# Autodesk Inventor assembly: functioning swerve drive
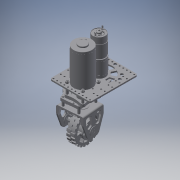
[picture p0: Inventor's stored thumbnail of the model, 180x180]
Saved by Autodesk Inventor 2019 (Build 230136000, 136)
## iProperties
Created: 2019-01-14
Part Number: functioning swerve drive
Document SubType Name: Assembly
Designer: josh
Author: josh
## Documents named in this file (35)
- D:\Synthesis Robots\Epsilon\Functioning swerve drive sub-assemblies\functioning swerve drive.iam
- D:\Synthesis Robots\Epsilon\Swerve drive parts\FR6ZZ-L Hex Bearing.ipt
- D:\Synthesis Robots\Epsilon\Swerve drive parts\375 Hex Output Shaft Rev 2.ipt
- D:\Synthesis Robots\Epsilon\Swerve drive parts\375 Hex Hub.ipt
- D:\Synthesis Robots\Epsilon\Swerve drive parts\10-24 Hex Washer Rolling x 3-4_93882A213.ipt
- D:\Synthesis Robots\Epsilon\Swerve drive parts\125x443 spacer SPS-0750-0443-0125.ipt
- D:\Synthesis Robots\Epsilon\Swerve drive parts\375 E-klip - Mcm 97431A320_97431A320.ipt
- D:\Synthesis Robots\Epsilon\Swerve drive parts\20t 1-25mod bevel gear.ipt
- D:\Synthesis Robots\Epsilon\Swerve drive parts\40t 1-25mod bevel gear.ipt
- D:\Synthesis Robots\Epsilon\Swerve drive parts\AMS C Housing Rev 2.ipt
- D:\Synthesis Robots\Epsilon\Swerve drive parts\10-32 Nylock Nut 1_90631A411.ipt
- D:\Synthesis Robots\Epsilon\Swerve drive parts\10-32x1250_shcs.ipt
- D:\Synthesis Robots\Epsilon\Swerve drive parts\620x215 alum spacer 83062 K-S.ipt
- D:\Synthesis Robots\Epsilon\Swerve drive parts\Bevel Input Shaft.ipt
- D:\Synthesis Robots\Epsilon\Swerve drive parts\FR8ZZ Bearing_smart.ipt
- D:\Synthesis Robots\Epsilon\Swerve drive parts\FR6ZZ Bearing_smart.ipt
- D:\Synthesis Robots\Epsilon\Swerve drive parts\12T CIM Shaft.ipt
- D:\Synthesis Robots\Epsilon\Swerve drive parts\Gear Plate.ipt
- D:\Synthesis Robots\Epsilon\Swerve drive parts\40T 20dp 375h_Inch - Spur gear 20DP 40T 14.5PA .372FW ---S40N3.0H2.0L0.25N.ipt
- D:\Synthesis Robots\Epsilon\Swerve drive parts\500 Washer am-1001.ipt
- D:\Synthesis Robots\Epsilon\Swerve drive parts\10-32x0625_shcs_HX-SHCS 0.19-32x1.375x1-C.ipt
- D:\Synthesis Robots\Epsilon\Swerve drive parts\1100x215 alum spacer 83062 K-S.ipt
- D:\Synthesis Robots\Epsilon\Swerve drive parts\10-32 Nylock Nut.ipt
- D:\Synthesis Robots\Epsilon\Swerve drive parts\10-32x1750_shcs_HX-SHCS 0.19-32x1.375x1-C.ipt
- D:\Synthesis Robots\Epsilon\Swerve drive parts\Bearing Plate.ipt
- D:\Synthesis Robots\Epsilon\Swerve drive parts\40T Sleeve Gear REV2.ipt
- D:\Synthesis Robots\Epsilon\Swerve drive parts\VEX 217-2736 0500 Collar Clamp.ipt
- D:\Synthesis Robots\Epsilon\Swerve drive parts\CIM Motor SW.ipt
- D:\Synthesis Robots\Epsilon\Swerve drive parts\Motor Mount Plate Rev 2.ipt
- D:\Synthesis Robots\Epsilon\Swerve drive parts\48T 10mm bore gear.ipt
- D:\Synthesis Robots\Epsilon\Swerve drive parts\PG-71.ipt
- D:\Synthesis Robots\Epsilon\Swerve drive parts\SHCS M4x10_91290A187.ipt
- D:\Synthesis Robots\Epsilon\Swerve drive parts\438x406 spacer 13RS100043.ipt
- D:\Synthesis Robots\Epsilon\Swerve drive parts\375 External Self Locking Ring_98430A134.ipt
- D:\Synthesis Robots\Epsilon\Swerve drive parts\4 in HiGrip Wheel.iam
## Components (68 placed, 34 different names)
1. FR6ZZ-L Hex Bearing:1
2. FR6ZZ-L Hex Bearing:2
3. 375 Hex Output Shaft Rev 2:1
4. 375 Hex Hub:1
5. 10-24 Hex Washer Rolling x 3-4_93882A213:1
6. 10-24 Hex Washer Rolling x 3-4_93882A213:2
7. 10-24 Hex Washer Rolling x 3-4_93882A213:3
8. 10-24 Hex Washer Rolling x 3-4_93882A213:4
9. 10-24 Hex Washer Rolling x 3-4_93882A213:5
10. 10-24 Hex Washer Rolling x 3-4_93882A213:6
11. 125x443 spacer SPS-0750-0443-0125:1
12. 375 E-klip - Mcm 97431A320_97431A320:1
13. 20t 1-25mod bevel gear:1
14. 40t 1-25mod bevel gear:1
15. AMS C Housing Rev 2:1
16. 10-32 Nylock Nut 1_90631A411:1
17. 10-32 Nylock Nut 1_90631A411:2
18. 10-32 Nylock Nut 1_90631A411:3
19. 10-32 Nylock Nut 1_90631A411:4
20. 10-32x1250_shcs:1
21. 10-32x1250_shcs:2
22. 10-32x1250_shcs:3
23. 10-32x1250_shcs:4
24. 620x215 alum spacer 83062 K-S:1
25. 620x215 alum spacer 83062 K-S:2
26. 620x215 alum spacer 83062 K-S:3
27. 620x215 alum spacer 83062 K-S:4
28. Bevel Input Shaft:1
29. FR8ZZ Bearing_smart:1
30. FR6ZZ Bearing_smart:1
31. 12T CIM Shaft:1
32. Gear Plate:1
33. 40T 20dp 375h_Inch - Spur gear 20DP 40T 14.5PA .372FW ---S40N3.0H2.0L0.25N:1
34. 500 Washer am-1001:1
35. 500 Washer am-1001:2
36. FR6ZZ Bearing_smart:2
37. 10-32x0625_shcs_HX-SHCS 0.19-32x1.375x1-C:1
38. 10-32x0625_shcs_HX-SHCS 0.19-32x1.375x1-C:2
39. 10-32x0625_shcs_HX-SHCS 0.19-32x1.375x1-C:3
40. 10-32x0625_shcs_HX-SHCS 0.19-32x1.375x1-C:4
41. 1100x215 alum spacer 83062 K-S:1
42. 10-32 Nylock Nut:1
43. 10-32x1750_shcs_HX-SHCS 0.19-32x1.375x1-C:1
44. 1100x215 alum spacer 83062 K-S:2
45. 1100x215 alum spacer 83062 K-S:3
46. 1100x215 alum spacer 83062 K-S:4
47. 10-32x1750_shcs_HX-SHCS 0.19-32x1.375x1-C:2
48. 10-32x1750_shcs_HX-SHCS 0.19-32x1.375x1-C:3
49. 10-32x1750_shcs_HX-SHCS 0.19-32x1.375x1-C:4
50. 10-32 Nylock Nut:2
51. 10-32 Nylock Nut:3
52. 10-32 Nylock Nut:4
53. Bearing Plate:1
54. 40T Sleeve Gear REV2:1
55. VEX 217-2736 0500 Collar Clamp:1
56. CIM Motor SW:1
57. Motor Mount Plate Rev 2:1
58. 48T 10mm bore gear:1
59. 10-32x0625_shcs_HX-SHCS 0.19-32x1.375x1-C:5
60. 10-32x0625_shcs_HX-SHCS 0.19-32x1.375x1-C:6
61. PG-71:1
62. SHCS M4x10_91290A187:1
63. SHCS M4x10_91290A187:2
64. SHCS M4x10_91290A187:3
65. SHCS M4x10_91290A187:4
66. 438x406 spacer 13RS100043:1
67. 375 External Self Locking Ring_98430A134:1
68. 4 in HiGrip Wheel:1 [sub-assembly]
## Relationships (145: Mate 125, Flush 11, RevoluteJoint 7, RelateRotation 2)
- [Mate]: 375 Hex Hub:1 ↔ 10-24 Hex Washer Rolling x 3-4_93882A213:6
- [Mate]: 375 Hex Hub:1 ↔ 10-24 Hex Washer Rolling x 3-4_93882A213:1
- [Mate]: 375 Hex Hub:1 ↔ 10-24 Hex Washer Rolling x 3-4_93882A213:5
- [Mate]: 375 Hex Hub:1 ↔ 10-24 Hex Washer Rolling x 3-4_93882A213:4
- [Mate]: 375 Hex Hub:1 ↔ 10-24 Hex Washer Rolling x 3-4_93882A213:3
- [Mate]: 375 Hex Hub:1 ↔ 10-24 Hex Washer Rolling x 3-4_93882A213:2
- [Mate]: 375 Hex Hub:1 ↔ 10-24 Hex Washer Rolling x 3-4_93882A213:2
- [Mate]: 375 Hex Hub:1 ↔ 10-24 Hex Washer Rolling x 3-4_93882A213:4
- [Mate]: 375 Hex Hub:1 ↔ 10-24 Hex Washer Rolling x 3-4_93882A213:3
- [Mate]: 375 Hex Hub:1 ↔ 10-24 Hex Washer Rolling x 3-4_93882A213:1
- [Mate]: 375 Hex Hub:1 ↔ 10-24 Hex Washer Rolling x 3-4_93882A213:6
- [Mate]: 375 Hex Hub:1 ↔ 10-24 Hex Washer Rolling x 3-4_93882A213:5
- [Mate]: 375 Hex Output Shaft Rev 2:1 ↔ 375 Hex Hub:1
- [Mate]: 375 Hex Output Shaft Rev 2:1 ↔ 375 Hex Hub:1
- [Mate]: FR6ZZ-L Hex Bearing:1 ↔ 375 Hex Output Shaft Rev 2:1
- [Mate]: FR6ZZ-L Hex Bearing:1 ↔ 375 Hex Output Shaft Rev 2:1
- [Mate]: 375 Hex Output Shaft Rev 2:1 ↔ 40t 1-25mod bevel gear:1
- [Mate]: 375 Hex Output Shaft Rev 2:1 ↔ 40t 1-25mod bevel gear:1
- [RevoluteJoint]: FR6ZZ-L Hex Bearing:2 ↔ AMS C Housing Rev 2:1
- [RevoluteJoint]: FR6ZZ-L Hex Bearing:1 ↔ AMS C Housing Rev 2:1
- [Mate]: FR6ZZ-L Hex Bearing:1 ↔ 125x443 spacer SPS-0750-0443-0125:1
- [Mate]: FR6ZZ-L Hex Bearing:1 ↔ 125x443 spacer SPS-0750-0443-0125:1
- [Mate]: 375 Hex Output Shaft Rev 2:1 ↔ 375 E-klip - Mcm 97431A320_97431A320:1
- [Mate]: 375 Hex Output Shaft Rev 2:1 ↔ 375 E-klip - Mcm 97431A320_97431A320:1
- [Mate]: 375 Hex Hub:1 ↔ 125x443 spacer SPS-0750-0443-0125:1
- [Flush]: FR6ZZ-L Hex Bearing:1 ↔ 375 Hex Output Shaft Rev 2:1
- [RevoluteJoint]: 10-32 Nylock Nut 1_90631A411:1 ↔ 10-32x1250_shcs:3
- [RevoluteJoint]: 10-32 Nylock Nut 1_90631A411:2 ↔ 10-32x1250_shcs:4
- [RevoluteJoint]: 10-32 Nylock Nut 1_90631A411:4 ↔ 10-32x1250_shcs:2
- [RevoluteJoint]: 10-32 Nylock Nut 1_90631A411:3 ↔ 10-32x1250_shcs:1
- [Mate]: 10-32x1250_shcs:2 ↔ Gear Plate:1
- [Mate]: 10-32x1250_shcs:2 ↔ 620x215 alum spacer 83062 K-S:2
- [Flush]: 10-32x1250_shcs:2 ↔ Gear Plate:1
- [Mate]: 620x215 alum spacer 83062 K-S:2 ↔ Gear Plate:1
- [Mate]: 10-32x1250_shcs:1 ↔ Gear Plate:1
- [Mate]: 10-32x1250_shcs:1 ↔ 620x215 alum spacer 83062 K-S:1
- [Flush]: 10-32x1250_shcs:1 ↔ Gear Plate:1
- [Mate]: 620x215 alum spacer 83062 K-S:1 ↔ Gear Plate:1
- [Mate]: 10-32x1250_shcs:3 ↔ Gear Plate:1
- [Flush]: 10-32x1250_shcs:3 ↔ Gear Plate:1
- [Mate]: 10-32x1250_shcs:3 ↔ 620x215 alum spacer 83062 K-S:3
- [Mate]: 620x215 alum spacer 83062 K-S:3 ↔ Gear Plate:1
- [Mate]: 10-32x1250_shcs:4 ↔ 620x215 alum spacer 83062 K-S:4
- [Flush]: 10-32x1250_shcs:4 ↔ Gear Plate:1
- [Mate]: 10-32x1250_shcs:4 ↔ Gear Plate:1
- [Mate]: 620x215 alum spacer 83062 K-S:4 ↔ Gear Plate:1
- [Mate]: FR8ZZ Bearing_smart:1 ↔ 12T CIM Shaft:1
- [Mate]: FR8ZZ Bearing_smart:1 ↔ 12T CIM Shaft:1
- [Mate]: 12T CIM Shaft:1 ↔ Gear Plate:1
- [Mate]: Bevel Input Shaft:1 ↔ FR6ZZ Bearing_smart:1
- [Mate]: Bevel Input Shaft:1 ↔ 500 Washer am-1001:1
- [Mate]: Bevel Input Shaft:1 ↔ 40T 20dp 375h_Inch - Spur gear 20DP 40T 14.5PA .372FW ---S40N3.0H2.0L0.25N:1
- [Mate]: Bevel Input Shaft:1 ↔ 40T 20dp 375h_Inch - Spur gear 20DP 40T 14.5PA .372FW ---S40N3.0H2.0L0.25N:1
- [Flush]: Bevel Input Shaft:1 ↔ 40T 20dp 375h_Inch - Spur gear 20DP 40T 14.5PA .372FW ---S40N3.0H2.0L0.25N:1
- [Mate]: Bevel Input Shaft:1 ↔ 500 Washer am-1001:2
- [Mate]: Bevel Input Shaft:1 ↔ FR6ZZ Bearing_smart:2
- [Mate]: 500 Washer am-1001:2 ↔ FR6ZZ Bearing_smart:2
- [Mate]: Bevel Input Shaft:1 ↔ 500 Washer am-1001:2
- [Flush]: Bevel Input Shaft:1 ↔ 500 Washer am-1001:1
- [Mate]: Gear Plate:1 ↔ FR6ZZ Bearing_smart:2
- [Mate]: Gear Plate:1 ↔ FR6ZZ Bearing_smart:2
- [RevoluteJoint]: 20t 1-25mod bevel gear:1 ↔ Bevel Input Shaft:1
- [Mate]: Gear Plate:1 ↔ 10-32x0625_shcs_HX-SHCS 0.19-32x1.375x1-C:3
- [Flush]: Gear Plate:1 ↔ 10-32x0625_shcs_HX-SHCS 0.19-32x1.375x1-C:3
- [Mate]: Gear Plate:1 ↔ 10-32x0625_shcs_HX-SHCS 0.19-32x1.375x1-C:2
- [Flush]: Gear Plate:1 ↔ 10-32x0625_shcs_HX-SHCS 0.19-32x1.375x1-C:2
- [Mate]: Gear Plate:1 ↔ 10-32x0625_shcs_HX-SHCS 0.19-32x1.375x1-C:1
- [Flush]: Gear Plate:1 ↔ 10-32x0625_shcs_HX-SHCS 0.19-32x1.375x1-C:1
- [Mate]: Gear Plate:1 ↔ 10-32x0625_shcs_HX-SHCS 0.19-32x1.375x1-C:4
- [Flush]: Gear Plate:1 ↔ 10-32x0625_shcs_HX-SHCS 0.19-32x1.375x1-C:4
- [Mate]: FR6ZZ Bearing_smart:1 ↔ 500 Washer am-1001:1
- [Mate]: AMS C Housing Rev 2:1 ↔ 10-32x1250_shcs:2
- [Mate]: AMS C Housing Rev 2:1 ↔ 10-32x1250_shcs:1
- [Mate]: AMS C Housing Rev 2:1 ↔ FR6ZZ Bearing_smart:1
- [Mate]: AMS C Housing Rev 2:1 ↔ FR8ZZ Bearing_smart:1
- [Mate]: 10-32x0625_shcs_HX-SHCS 0.19-32x1.375x1-C:3 ↔ 40T Sleeve Gear REV2:1
- [Mate]: 10-32x0625_shcs_HX-SHCS 0.19-32x1.375x1-C:4 ↔ 40T Sleeve Gear REV2:1
- [Mate]: 10-32x0625_shcs_HX-SHCS 0.19-32x1.375x1-C:1 ↔ 40T Sleeve Gear REV2:1
- [Mate]: 10-32x0625_shcs_HX-SHCS 0.19-32x1.375x1-C:2 ↔ 40T Sleeve Gear REV2:1
- [Mate]: 12T CIM Shaft:1 ↔ 40T Sleeve Gear REV2:1
- [Mate]: Gear Plate:1 ↔ 40T Sleeve Gear REV2:1
- [Mate]: 10-32 Nylock Nut:1 ↔ 10-32x1750_shcs_HX-SHCS 0.19-32x1.375x1-C:1
- [Mate]: 10-32x1750_shcs_HX-SHCS 0.19-32x1.375x1-C:4 ↔ 10-32 Nylock Nut:2
- [Mate]: 10-32x1750_shcs_HX-SHCS 0.19-32x1.375x1-C:3 ↔ 10-32 Nylock Nut:4
- [Mate]: 10-32x1750_shcs_HX-SHCS 0.19-32x1.375x1-C:2 ↔ 10-32 Nylock Nut:3
- [Mate]: 1100x215 alum spacer 83062 K-S:3 ↔ 10-32x1750_shcs_HX-SHCS 0.19-32x1.375x1-C:3
- [Mate]: 10-32x1750_shcs_HX-SHCS 0.19-32x1.375x1-C:3 ↔ Bearing Plate:1
- [Mate]: 10-32x1750_shcs_HX-SHCS 0.19-32x1.375x1-C:3 ↔ Bearing Plate:1
- [Mate]: 1100x215 alum spacer 83062 K-S:2 ↔ 10-32x1750_shcs_HX-SHCS 0.19-32x1.375x1-C:4
- [Mate]: 10-32x1750_shcs_HX-SHCS 0.19-32x1.375x1-C:4 ↔ Bearing Plate:1
- [Mate]: 1100x215 alum spacer 83062 K-S:2 ↔ Bearing Plate:1
- [Mate]: 10-32x1750_shcs_HX-SHCS 0.19-32x1.375x1-C:4 ↔ Bearing Plate:1
- [Mate]: 10-32 Nylock Nut:2 ↔ Motor Mount Plate Rev 2:1
- [Mate]: 1100x215 alum spacer 83062 K-S:3 ↔ Bearing Plate:1
- [Mate]: 10-32 Nylock Nut:4 ↔ Motor Mount Plate Rev 2:1
- [Mate]: 10-32x1750_shcs_HX-SHCS 0.19-32x1.375x1-C:1 ↔ Bearing Plate:1
- [Mate]: 10-32 Nylock Nut:1 ↔ 10-32x1750_shcs_HX-SHCS 0.19-32x1.375x1-C:1
- [Mate]: 10-32 Nylock Nut:1 ↔ Motor Mount Plate Rev 2:1
- [Mate]: 10-32x1750_shcs_HX-SHCS 0.19-32x1.375x1-C:1 ↔ Bearing Plate:1
- [Mate]: 1100x215 alum spacer 83062 K-S:1 ↔ 10-32x1750_shcs_HX-SHCS 0.19-32x1.375x1-C:1
- [Mate]: 1100x215 alum spacer 83062 K-S:1 ↔ Bearing Plate:1
- [Mate]: 10-32x1750_shcs_HX-SHCS 0.19-32x1.375x1-C:2 ↔ Bearing Plate:1
- [Mate]: 10-32x1750_shcs_HX-SHCS 0.19-32x1.375x1-C:2 ↔ Bearing Plate:1
- [Mate]: 1100x215 alum spacer 83062 K-S:4 ↔ 10-32x1750_shcs_HX-SHCS 0.19-32x1.375x1-C:2
- [Mate]: 1100x215 alum spacer 83062 K-S:4 ↔ Bearing Plate:1
- [Mate]: 10-32 Nylock Nut:3 ↔ Motor Mount Plate Rev 2:1
- [Mate]: CIM Motor SW:1 ↔ 10-32x0625_shcs_HX-SHCS 0.19-32x1.375x1-C:6
- [Mate]: Motor Mount Plate Rev 2:1 ↔ 10-32x0625_shcs_HX-SHCS 0.19-32x1.375x1-C:6
- [Mate]: Motor Mount Plate Rev 2:1 ↔ 10-32x0625_shcs_HX-SHCS 0.19-32x1.375x1-C:6
- [Mate]: CIM Motor SW:1 ↔ 10-32x0625_shcs_HX-SHCS 0.19-32x1.375x1-C:5
- [Mate]: Motor Mount Plate Rev 2:1 ↔ 10-32x0625_shcs_HX-SHCS 0.19-32x1.375x1-C:5
- [Mate]: Motor Mount Plate Rev 2:1 ↔ 10-32x0625_shcs_HX-SHCS 0.19-32x1.375x1-C:5
- [Mate]: 12T CIM Shaft:1 ↔ CIM Motor SW:1
- [Mate]: VEX 217-2736 0500 Collar Clamp:1 ↔ CIM Motor SW:1
- [Mate]: VEX 217-2736 0500 Collar Clamp:1 ↔ Motor Mount Plate Rev 2:1
- [Mate]: 12T CIM Shaft:1 ↔ CIM Motor SW:1
- [Mate]: CIM Motor SW:1 ↔ Motor Mount Plate Rev 2:1
- [Mate]: PG-71:1 ↔ 375 External Self Locking Ring_98430A134:1
- [Mate]: 48T 10mm bore gear:1 ↔ PG-71:1
- [Mate]: 10-32x1750_shcs_HX-SHCS 0.19-32x1.375x1-C:1 ↔ Motor Mount Plate Rev 2:1
- [Mate]: 10-32x1750_shcs_HX-SHCS 0.19-32x1.375x1-C:4 ↔ Motor Mount Plate Rev 2:1
- [Mate]: 1100x215 alum spacer 83062 K-S:1 ↔ Motor Mount Plate Rev 2:1
- [Mate]: PG-71:1 ↔ 438x406 spacer 13RS100043:1
- [Mate]: Motor Mount Plate Rev 2:1 ↔ 438x406 spacer 13RS100043:1
- [Mate]: Motor Mount Plate Rev 2:1 ↔ SHCS M4x10_91290A187:2
- [Mate]: Motor Mount Plate Rev 2:1 ↔ SHCS M4x10_91290A187:1
- [Mate]: Motor Mount Plate Rev 2:1 ↔ SHCS M4x10_91290A187:4
- [Mate]: Motor Mount Plate Rev 2:1 ↔ SHCS M4x10_91290A187:3
- [Mate]: Motor Mount Plate Rev 2:1 ↔ SHCS M4x10_91290A187:1
- [Mate]: Motor Mount Plate Rev 2:1 ↔ SHCS M4x10_91290A187:2
- [Mate]: Motor Mount Plate Rev 2:1 ↔ SHCS M4x10_91290A187:4
- [Mate]: Motor Mount Plate Rev 2:1 ↔ SHCS M4x10_91290A187:3
- [Mate]: PG-71:1 ↔ 438x406 spacer 13RS100043:1
- [Mate]: Motor Mount Plate Rev 2:1 ↔ PG-71:1
- [Mate]: 48T 10mm bore gear:1 ↔ 438x406 spacer 13RS100043:1
- [Mate]: PG-71:1 ↔ 375 External Self Locking Ring_98430A134:1
- [RelateRotation] (1 ul): 20t 1-25mod bevel gear:1 ↔ 40t 1-25mod bevel gear:1
- [Mate]: 20t 1-25mod bevel gear:1 ↔ Bevel Input Shaft:1
- [RelateRotation] (1 ul): 40T Sleeve Gear REV2:1 ↔ 48T 10mm bore gear:1
- [Mate]: 48T 10mm bore gear:1 ↔ PG-71:1
- [Mate]: 10-24 Hex Washer Rolling x 3-4_93882A213:6 ↔ 4 in HiGrip Wheel:1
- [Mate]: 10-24 Hex Washer Rolling x 3-4_93882A213:5 ↔ 4 in HiGrip Wheel:1
- [Mate]: 10-24 Hex Washer Rolling x 3-4_93882A213:4 ↔ 4 in HiGrip Wheel:1
- [Mate]: 375 Hex Hub:1 ↔ 4 in HiGrip Wheel:1
- [Mate]: 40t 1-25mod bevel gear:1 ↔ 4 in HiGrip Wheel:1
## Named parameters: d291_d98_d143 = 0 mm, d292_d99_d144 = 150.286815 deg, d293_d100_d146 = 0 mm, d294_d101_d147 = 0 mm, d295_d102_d148 = 0 mm, d296_d103_d149 = 0 mm, d297_d104_d150 = 0 mm, d298_d122_d151 = 0 mm, d299_d123_d152 = 0 mm, d300_d124_d153 = 0 mm, d301_d125_d154 = 0 mm, d302_d126_d155 = 0 mm, d303_d127_d156 = 0 mm, d304_d128_d157 = 0 mm, d305_d129_d158 = 0 mm, d306_d130_d159 = 0 mm, d307_d131_d160 = 0 mm, d308_d132_d161 = 0 mm, d309_d133_d165 = 0 mm, d310_d102 = 0 mm, d311_d103 = 0 mm, d312_d104 = 0 mm, d313_d105 = 0 mm, d314_d106 = 0 mm, d315_d107 = 0 mm, d316_d108 = 0 mm, d317_d109 = 0 mm, d318_d110 = 0 mm, d319_d113 = 0 mm, d320_d114 = 0 mm, d321_d117 = 0 mm, d322_d118 = 74.365012 deg, d323_d119 = 0 mm, d324_d120 = -54.363492 deg, d325_d121 = 0 mm, d326_d122 = 0 mm, d327_d131 = 0 mm, d328_d132 = 0 mm, d329_d135 = 0 mm, d330_d136 = 0 mm, d331_d137 = 0 mm, d332_d138 = -163.765471 deg, d333_d95 = 0 mm, d334_d96 = 0 mm, d335_d97 = 0 mm, d336_d98 = 0 mm, d337_d99 = 0 mm, d338_d100 = 0 mm, d339_d101 = 0 mm, d340_d163 = 0 mm, d341_d126 = 0 mm, d342_d127 = 0 mm, d343_d128 = 0 mm, d344_d129 = 0 mm, d345_d162 = 0 mm, d346_d777 = 0 mm, d347_d778 = 1, d348_d776 = 1, d349_d263 = 0 mm, d350_d264 = 0 mm, d351_d266 = 0 mm, d352_d267 = 0 mm, d353_d268 = 0 mm, d354_d270 = 0 mm, d355_d271 = 0 mm, d356_d272 = 0 mm, d357_d273 = 0 mm, d358_d274 = 0 mm, d359_d275 = 0 mm, d360_d276 = 0 mm, d361_d277 = 0 mm, d362_d278 = 0 mm, d363_d279 = 0 mm, d364_d280 = 0 mm, d365_d232 = 0 mm, d366_d233 = 0 mm, d367_d234 = 0 mm, d368_d235 = 0 mm, d369_d236 = 0 mm, d370_d237 = 0 mm, d371_d238 = 0 mm, d372_d239 = 0 mm, d373_d240 = 0 mm, d374_d241 = 0 mm, d375_d242 = 0 mm, d376_d243 = 0 mm, d377_d244 = 0 mm, d378_d245 = 0 mm, d379_d246 = 0 mm, d380_d247 = 0 mm, d381_d248 = 0 mm, d383_d253 = 0 mm, d384_d254 = 0 mm, d385_d255 = 0 mm, d386_d256 = 0 mm, d387_d257 = 0 mm, d388_d258 = 0 mm, d389_d259 = 0 mm, d390_d262 = 0 mm, d391_d199 = 0 mm, d392_d200 = 0 mm, d393_d201 = 0 mm, d394_d202 = 0 mm, d395_d203 = 0 mm, d396_d204 = 0 mm, d397_d206 = 0 mm, d398_d207 = 0 mm, d399_d209 = 0 mm, d400_d210 = 0 mm, d401_d211 = 0 mm, d402_d212 = 0 mm, d403_d213 = 0 mm, d404_d214 = 0 mm, d405_d215 = 0 mm, d406_d216 = 0 mm, d407_d217 = 0 mm, d408_d218 = 0 mm, d409_d219 = 0 mm, d170_d220 = 0 mm, d171_d221 = 0 mm, d174_d222 = 0 mm, d175_d223 = 0 mm, d176_d224 = 0 mm, d177_d225 = 0 mm, d178_d226 = 0 mm, d180_d227 = 0 mm, d181_d228 = 0 mm, d182_d229 = 0 mm, d183_d230 = 0 mm, d188_d231 = 0 mm, d189_d93_d166 = 0 mm, d193_d94_d167 = 0 mm, d196_d95_d168 = 0 mm, d205_d96_d169 = 0 mm, d208_d172 = 0 mm, d250_d173 = 0 mm, d251_d179 = 0 mm, d252_d184 = 0 mm, d260_d185 = 0 mm, d261_d186 = 0 mm, d265_d187 = 0 mm, d269_d190 = 0 mm, d281_d191 = 0 mm, d282_d192 = 0 mm, d283_d194 = 0 mm, d284_d195 = -120 deg, d285_d197 = 0 mm, d286_d198 = 0 mm, d287_d94_d139 = 0 mm, d288_d95_d140 = -154.263513 deg, d289_d96_d141 = 0 mm, d290_d97_d142 = 63.496867 deg
